# Autodesk Inventor assembly: HCMUTE-CDT23-PLXR_KHUNG
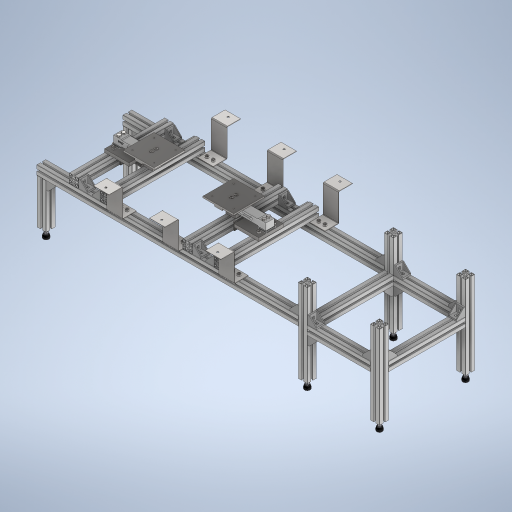
[picture p0: Inventor's stored thumbnail of the model, 512x512]
Saved by Autodesk Inventor 2023 (Build 270158000, 158)
## iProperties
Created: 2023-11-19
Part Number: HCMUTE-CDT23-PLXR_KHUNG
Document SubType Name: Assembly
Designer: havie
Mass: 52555 g
Surface Area: 83477.5 cm^2
Volume: 13075.1 cm^3
Density: 4.01946 g/cm^3
Author: havie
## Documents named in this file (13)
- D:\DO_AN_CDT\1.1. PART\HCMUTE-CDT23-PLXR_KHUNG.iam
- D:\DO_AN_CDT\1.1. PART\HCMUTE-CDT23-FRAME_ASEMBLY.iam
- C:\Users\havie\Documents\Inventor\Content Center Files\R2023\en-US\ISO 4762(2)\ISO 4762 - M6 x 16ISO.ipt
- C:\Users\havie\Documents\Inventor\Content Center Files\R2023\en-US\ISO 4762(2)\ISO 4762 - M6 x 25ISO.ipt
- D:\DO_AN_CDT\1.1. PART\HCMUTE-CDT23-LOADCELL.ipt
- D:\DO_AN_CDT\1.1. PART\HCMUTE-CDT23-DE_CHEM_LOADCELL.ipt
- D:\DO_AN_CDT\1.1. PART\HCMUTE-CDT23-DE_GA_LOADCELL.ipt
- D:\DO_AN_CDT\1.1. PART\HCMUTE-CDT23-GOI_CHONG_QTAI.ipt
- D:\DO_AN_CDT\1.1. PART\HCMUTE-CDT23-GOI_DO.ipt
- C:\Users\havie\Documents\Inventor\Content Center Files\R2023\en-US\ISO 4017(1)\ISO 4017 - M6 x 45 - ISO.ipt
- C:\Users\havie\Documents\Inventor\Content Center Files\R2023\en-US\ISO 4762(2)\ISO 4762 - M6 x 10ISO.ipt
- D:\DO_AN_CDT\1.1. PART\HCMUTE-CDT23-BAN_CAN_LOADCELL.ipt
- D:\DO_AN_CDT\1.1. PART\HCMUTE-CDT23-KXL_CHAN-GA.ipt
## Components (53 placed, 12 different names)
1. HCMUTE-CDT23-FRAME_ASEMBLY:1 [sub-assembly] — Mate:84, Flush:8, Flush:9, Mate:92, Flush:12, Mate:102, Flush:13, Mate:152, Flush:16, Mate:153, Flush:18, Mate:154, Flush:20, Mate:276, Flush:52, Mate:277, Mate:282, Mate:283, Mate:284, Mate:285, Mate:320, Flush:63, Mate:321, Mate:322, Mate:323
2. HCMUTE-CDT23-LOADCELL:1 — Mate:88, Mate:89, Mate:90, Mate:94, Mate:95, Mate:96, Mate:97, Flush:14, Mate:113, Mate:114, Mate:115
3. HCMUTE-CDT23-DE_CHEM_LOADCELL:1 — Mate:85, Mate:86, Mate:87, Mate:88, Mate:89, Mate:90
4. HCMUTE-CDT23-DE_GA_LOADCELL:1 — Mate:84, Flush:8, Flush:9, Mate:85, Mate:86, Mate:87, Mate:93, Mate:98, Mate:99, Mate:100, Mate:101, Flush:19
5. HCMUTE-CDT23-GOI_CHONG_QTAI:1 — Mate:102, Flush:13, Mate:103, Mate:104, Flush:14
6. HCMUTE-CDT23-GOI_DO:1 — Mate:92, Flush:12, Mate:93, Mate:105, Mate:106, Mate:107, Mate:108, Mate:109, Mate:110, Mate:111, Mate:112, Flush:17
7. ISO 4017 M6 x 45:1 — Mate:94, Mate:97
8. ISO 4017 M6 x 45:2 — Mate:95, Mate:96
9. ISO 4762 M6 x 16:31 — Mate:100, Mate:101
10. ISO 4762 M6 x 16:33 — Mate:98, Mate:99
11. ISO 4762 M6 x 16:34 — Mate:103, Mate:104
12. ISO 4762 M6 x 10:1 — Mate:105, Mate:106
13. ISO 4762 M6 x 10:2 — Mate:111, Mate:112
14. ISO 4762 M6 x 10:3 — Mate:109, Mate:110
15. ISO 4762 M6 x 10:4 — Mate:107, Mate:108
16. HCMUTE-CDT23-BAN_CAN_LOADCELL:1 — Mate:113, Mate:114, Mate:115, Mate:116, Mate:117, Mate:118, Mate:119
17. ISO 4762 M6 x 25:5 — Mate:116, Mate:118
18. ISO 4762 M6 x 25:6 — Mate:117, Mate:119
19. HCMUTE-CDT23-LOADCELL:2 — Flush:21
20. HCMUTE-CDT23-DE_CHEM_LOADCELL:2
21. HCMUTE-CDT23-DE_GA_LOADCELL:2 — Mate:153, Flush:18, Flush:19
22. HCMUTE-CDT23-GOI_CHONG_QTAI:2 — Mate:154, Flush:20, Flush:21
23. HCMUTE-CDT23-GOI_DO:2 — Mate:152, Flush:16, Flush:17
24. ISO 4017 M6 x 45:3
25. ISO 4017 M6 x 45:4
26. ISO 4762 M6 x 16:35
27. ISO 4762 M6 x 16:36
28. ISO 4762 M6 x 16:37
29. ISO 4762 M6 x 10:5
30. ISO 4762 M6 x 10:6
31. ISO 4762 M6 x 10:7
32. ISO 4762 M6 x 10:8
33. HCMUTE-CDT23-BAN_CAN_LOADCELL:2
34. ISO 4762 M6 x 25:7
35. ISO 4762 M6 x 25:8
36. HCMUTE-CDT23-KXL_CHAN-GA:1 — Mate:276, Flush:52, Mate:277, Mate:278, Mate:279, Mate:280, Mate:281, Flush:53
37. HCMUTE-CDT23-KXL_CHAN-GA:2 — Mate:282, Mate:283, Flush:53, Flush:54, Flush:65
38. HCMUTE-CDT23-KXL_CHAN-GA:3 — Mate:284, Mate:285, Flush:54, Flush:67
39. HCMUTE-CDT23-KXL_CHAN-GA:4 — Mate:320, Flush:63, Mate:321, Flush:64, Flush:66
40. HCMUTE-CDT23-KXL_CHAN-GA:5 — Mate:322, Flush:64, Flush:65
41. HCMUTE-CDT23-KXL_CHAN-GA:6 — Mate:323, Flush:66, Flush:67, Mate:327, Mate:328, Mate:329, Mate:330
42. ISO 4762 M6 x 10:9 — Mate:280, Mate:281
43. ISO 4762 M6 x 10:10 — Mate:278, Mate:279
44. ISO 4762 M6 x 10:11
45. ISO 4762 M6 x 10:12
46. ISO 4762 M6 x 10:13
47. ISO 4762 M6 x 10:14
48. ISO 4762 M6 x 10:16 — Mate:329, Mate:330
49. ISO 4762 M6 x 10:15 — Mate:327, Mate:328
50. ISO 4762 M6 x 10:17
51. ISO 4762 M6 x 10:18
52. ISO 4762 M6 x 10:19
53. ISO 4762 M6 x 10:20
## Component patterns: (3 elements, first: ISO 4762 M6 x 10:9 + ISO 4762 M6 x 10:10), (3 elements, first: ISO 4762 M6 x 10:16 + ISO 4762 M6 x 10:15)
## Relationships (111: Mate 89, Flush 20, Symmetry 2)
- Mate:84: HCMUTE-CDT23-FRAME_ASEMBLY:1 ↔ HCMUTE-CDT23-DE_GA_LOADCELL:1
- Flush:8: HCMUTE-CDT23-FRAME_ASEMBLY:1 ↔ HCMUTE-CDT23-DE_GA_LOADCELL:1
- Flush:9 (115 mm): HCMUTE-CDT23-FRAME_ASEMBLY:1 ↔ HCMUTE-CDT23-DE_GA_LOADCELL:1
- Mate:85: HCMUTE-CDT23-DE_CHEM_LOADCELL:1 ↔ HCMUTE-CDT23-DE_GA_LOADCELL:1
- Mate:86: HCMUTE-CDT23-DE_CHEM_LOADCELL:1 ↔ HCMUTE-CDT23-DE_GA_LOADCELL:1
- Mate:87: HCMUTE-CDT23-DE_CHEM_LOADCELL:1 ↔ HCMUTE-CDT23-DE_GA_LOADCELL:1
- Mate:88: HCMUTE-CDT23-LOADCELL:1 ↔ HCMUTE-CDT23-DE_CHEM_LOADCELL:1
- Mate:89: HCMUTE-CDT23-LOADCELL:1 ↔ HCMUTE-CDT23-DE_CHEM_LOADCELL:1
- Mate:90: HCMUTE-CDT23-LOADCELL:1 ↔ HCMUTE-CDT23-DE_CHEM_LOADCELL:1
- Mate:92: HCMUTE-CDT23-FRAME_ASEMBLY:1 ↔ HCMUTE-CDT23-GOI_DO:1
- Flush:12: HCMUTE-CDT23-FRAME_ASEMBLY:1 ↔ HCMUTE-CDT23-GOI_DO:1
- Mate:93: HCMUTE-CDT23-DE_GA_LOADCELL:1 ↔ HCMUTE-CDT23-GOI_DO:1
- Mate:94: HCMUTE-CDT23-LOADCELL:1 ↔ ISO 4017 M6 x 45:1
- Mate:95: HCMUTE-CDT23-LOADCELL:1 ↔ ISO 4017 M6 x 45:2
- Mate:96: HCMUTE-CDT23-LOADCELL:1 ↔ ISO 4017 M6 x 45:2
- Mate:97: HCMUTE-CDT23-LOADCELL:1 ↔ ISO 4017 M6 x 45:1
- Mate:98: HCMUTE-CDT23-DE_GA_LOADCELL:1 ↔ ISO 4762 M6 x 16:33
- Mate:99: HCMUTE-CDT23-DE_GA_LOADCELL:1 ↔ ISO 4762 M6 x 16:33
- Mate:100: HCMUTE-CDT23-DE_GA_LOADCELL:1 ↔ ISO 4762 M6 x 16:31
- Mate:101: HCMUTE-CDT23-DE_GA_LOADCELL:1 ↔ ISO 4762 M6 x 16:31
- Mate:102: HCMUTE-CDT23-FRAME_ASEMBLY:1 ↔ HCMUTE-CDT23-GOI_CHONG_QTAI:1
- Flush:13: HCMUTE-CDT23-FRAME_ASEMBLY:1 ↔ HCMUTE-CDT23-GOI_CHONG_QTAI:1
- Mate:103: HCMUTE-CDT23-GOI_CHONG_QTAI:1 ↔ ISO 4762 M6 x 16:34
- Mate:104: HCMUTE-CDT23-GOI_CHONG_QTAI:1 ↔ ISO 4762 M6 x 16:34
- Flush:14 (-1.5 mm): HCMUTE-CDT23-LOADCELL:1 ↔ HCMUTE-CDT23-GOI_CHONG_QTAI:1
- Mate:105: HCMUTE-CDT23-GOI_DO:1 ↔ ISO 4762 M6 x 10:1
- Mate:106: HCMUTE-CDT23-GOI_DO:1 ↔ ISO 4762 M6 x 10:1
- Mate:107: HCMUTE-CDT23-GOI_DO:1 ↔ ISO 4762 M6 x 10:4
- Mate:108: HCMUTE-CDT23-GOI_DO:1 ↔ ISO 4762 M6 x 10:4
- Mate:109: HCMUTE-CDT23-GOI_DO:1 ↔ ISO 4762 M6 x 10:3
- Mate:110: HCMUTE-CDT23-GOI_DO:1 ↔ ISO 4762 M6 x 10:3
- Mate:111: HCMUTE-CDT23-GOI_DO:1 ↔ ISO 4762 M6 x 10:2
- Mate:112: HCMUTE-CDT23-GOI_DO:1 ↔ ISO 4762 M6 x 10:2
- Mate:113: HCMUTE-CDT23-LOADCELL:1 ↔ HCMUTE-CDT23-BAN_CAN_LOADCELL:1
- Mate:114: HCMUTE-CDT23-LOADCELL:1 ↔ HCMUTE-CDT23-BAN_CAN_LOADCELL:1
- Mate:115: HCMUTE-CDT23-LOADCELL:1 ↔ HCMUTE-CDT23-BAN_CAN_LOADCELL:1
- Mate:116: HCMUTE-CDT23-BAN_CAN_LOADCELL:1 ↔ ISO 4762 M6 x 25:5
- Mate:117: HCMUTE-CDT23-BAN_CAN_LOADCELL:1 ↔ ISO 4762 M6 x 25:6
- Mate:118: HCMUTE-CDT23-BAN_CAN_LOADCELL:1 ↔ ISO 4762 M6 x 25:5
- Mate:119: HCMUTE-CDT23-BAN_CAN_LOADCELL:1 ↔ ISO 4762 M6 x 25:6
- [Mate]: HCMUTE-CDT23-DE_CHEM_LOADCELL:2 ↔ HCMUTE-CDT23-DE_GA_LOADCELL:2
- [Mate]: HCMUTE-CDT23-DE_CHEM_LOADCELL:2 ↔ HCMUTE-CDT23-DE_GA_LOADCELL:2
- [Mate]: HCMUTE-CDT23-DE_CHEM_LOADCELL:2 ↔ HCMUTE-CDT23-DE_GA_LOADCELL:2
- [Mate]: HCMUTE-CDT23-LOADCELL:2 ↔ HCMUTE-CDT23-DE_CHEM_LOADCELL:2
- [Mate]: HCMUTE-CDT23-LOADCELL:2 ↔ HCMUTE-CDT23-DE_CHEM_LOADCELL:2
- [Mate]: HCMUTE-CDT23-LOADCELL:2 ↔ HCMUTE-CDT23-DE_CHEM_LOADCELL:2
- [Mate]: HCMUTE-CDT23-DE_GA_LOADCELL:2 ↔ HCMUTE-CDT23-GOI_DO:2
- [Mate]: HCMUTE-CDT23-LOADCELL:2 ↔ ISO 4017 M6 x 45:3
- [Mate]: HCMUTE-CDT23-LOADCELL:2 ↔ ISO 4017 M6 x 45:4
- [Mate]: HCMUTE-CDT23-LOADCELL:2 ↔ ISO 4017 M6 x 45:4
- [Mate]: HCMUTE-CDT23-LOADCELL:2 ↔ ISO 4017 M6 x 45:3
- [Mate]: HCMUTE-CDT23-DE_GA_LOADCELL:2 ↔ ISO 4762 M6 x 16:36
- [Mate]: HCMUTE-CDT23-DE_GA_LOADCELL:2 ↔ ISO 4762 M6 x 16:36
- [Mate]: HCMUTE-CDT23-DE_GA_LOADCELL:2 ↔ ISO 4762 M6 x 16:35
- [Mate]: HCMUTE-CDT23-DE_GA_LOADCELL:2 ↔ ISO 4762 M6 x 16:35
- [Mate]: HCMUTE-CDT23-GOI_CHONG_QTAI:2 ↔ ISO 4762 M6 x 16:37
- [Mate]: HCMUTE-CDT23-GOI_CHONG_QTAI:2 ↔ ISO 4762 M6 x 16:37
- [Flush] (-1.5 mm): HCMUTE-CDT23-LOADCELL:2 ↔ HCMUTE-CDT23-GOI_CHONG_QTAI:2
- [Mate]: HCMUTE-CDT23-GOI_DO:2 ↔ ISO 4762 M6 x 10:5
- [Mate]: HCMUTE-CDT23-GOI_DO:2 ↔ ISO 4762 M6 x 10:5
- [Mate]: HCMUTE-CDT23-GOI_DO:2 ↔ ISO 4762 M6 x 10:8
- [Mate]: HCMUTE-CDT23-GOI_DO:2 ↔ ISO 4762 M6 x 10:8
- [Mate]: HCMUTE-CDT23-GOI_DO:2 ↔ ISO 4762 M6 x 10:7
- [Mate]: HCMUTE-CDT23-GOI_DO:2 ↔ ISO 4762 M6 x 10:7
- [Mate]: HCMUTE-CDT23-GOI_DO:2 ↔ ISO 4762 M6 x 10:6
- [Mate]: HCMUTE-CDT23-GOI_DO:2 ↔ ISO 4762 M6 x 10:6
- [Mate]: HCMUTE-CDT23-LOADCELL:2 ↔ HCMUTE-CDT23-BAN_CAN_LOADCELL:2
- [Mate]: HCMUTE-CDT23-LOADCELL:2 ↔ HCMUTE-CDT23-BAN_CAN_LOADCELL:2
- [Mate]: HCMUTE-CDT23-LOADCELL:2 ↔ HCMUTE-CDT23-BAN_CAN_LOADCELL:2
- [Mate]: HCMUTE-CDT23-BAN_CAN_LOADCELL:2 ↔ ISO 4762 M6 x 25:7
- [Mate]: HCMUTE-CDT23-BAN_CAN_LOADCELL:2 ↔ ISO 4762 M6 x 25:8
- [Mate]: HCMUTE-CDT23-BAN_CAN_LOADCELL:2 ↔ ISO 4762 M6 x 25:7
- [Mate]: HCMUTE-CDT23-BAN_CAN_LOADCELL:2 ↔ ISO 4762 M6 x 25:8
- Mate:152: HCMUTE-CDT23-FRAME_ASEMBLY:1 ↔ HCMUTE-CDT23-GOI_DO:2
- Flush:16: HCMUTE-CDT23-FRAME_ASEMBLY:1 ↔ HCMUTE-CDT23-GOI_DO:2
- Flush:17: HCMUTE-CDT23-GOI_DO:1 ↔ HCMUTE-CDT23-GOI_DO:2
- Mate:153: HCMUTE-CDT23-FRAME_ASEMBLY:1 ↔ HCMUTE-CDT23-DE_GA_LOADCELL:2
- Flush:18: HCMUTE-CDT23-FRAME_ASEMBLY:1 ↔ HCMUTE-CDT23-DE_GA_LOADCELL:2
- Flush:19: HCMUTE-CDT23-DE_GA_LOADCELL:1 ↔ HCMUTE-CDT23-DE_GA_LOADCELL:2
- Mate:154: HCMUTE-CDT23-FRAME_ASEMBLY:1 ↔ HCMUTE-CDT23-GOI_CHONG_QTAI:2
- Flush:20: HCMUTE-CDT23-FRAME_ASEMBLY:1 ↔ HCMUTE-CDT23-GOI_CHONG_QTAI:2
- Flush:21 (-1.5 mm): HCMUTE-CDT23-LOADCELL:2 ↔ HCMUTE-CDT23-GOI_CHONG_QTAI:2
- Symmetry:1
- Symmetry:2
- Mate:235
- Mate:276: HCMUTE-CDT23-FRAME_ASEMBLY:1 ↔ HCMUTE-CDT23-KXL_CHAN-GA:1
- Flush:52 (-15 mm): HCMUTE-CDT23-FRAME_ASEMBLY:1 ↔ HCMUTE-CDT23-KXL_CHAN-GA:1
- Mate:277: HCMUTE-CDT23-FRAME_ASEMBLY:1 ↔ HCMUTE-CDT23-KXL_CHAN-GA:1
- Mate:278: HCMUTE-CDT23-KXL_CHAN-GA:1 ↔ ISO 4762 M6 x 10:10
- Mate:279: HCMUTE-CDT23-KXL_CHAN-GA:1 ↔ ISO 4762 M6 x 10:10
- Mate:280: HCMUTE-CDT23-KXL_CHAN-GA:1 ↔ ISO 4762 M6 x 10:9
- Mate:281: HCMUTE-CDT23-KXL_CHAN-GA:1 ↔ ISO 4762 M6 x 10:9
- Mate:282: HCMUTE-CDT23-FRAME_ASEMBLY:1 ↔ HCMUTE-CDT23-KXL_CHAN-GA:2
- Mate:283: HCMUTE-CDT23-FRAME_ASEMBLY:1 ↔ HCMUTE-CDT23-KXL_CHAN-GA:2
- Flush:53: HCMUTE-CDT23-KXL_CHAN-GA:1 ↔ HCMUTE-CDT23-KXL_CHAN-GA:2
- Mate:284 (6 mm): HCMUTE-CDT23-FRAME_ASEMBLY:1 ↔ HCMUTE-CDT23-KXL_CHAN-GA:3
- Mate:285: HCMUTE-CDT23-FRAME_ASEMBLY:1 ↔ HCMUTE-CDT23-KXL_CHAN-GA:3
- Flush:54: HCMUTE-CDT23-KXL_CHAN-GA:2 ↔ HCMUTE-CDT23-KXL_CHAN-GA:3
- Mate:320: HCMUTE-CDT23-FRAME_ASEMBLY:1 ↔ HCMUTE-CDT23-KXL_CHAN-GA:4
- Flush:63 (-16 mm): HCMUTE-CDT23-FRAME_ASEMBLY:1 ↔ HCMUTE-CDT23-KXL_CHAN-GA:4
- Mate:321: HCMUTE-CDT23-FRAME_ASEMBLY:1 ↔ HCMUTE-CDT23-KXL_CHAN-GA:4
- Mate:322: HCMUTE-CDT23-FRAME_ASEMBLY:1 ↔ HCMUTE-CDT23-KXL_CHAN-GA:5
- Flush:64: HCMUTE-CDT23-KXL_CHAN-GA:4 ↔ HCMUTE-CDT23-KXL_CHAN-GA:5
- Flush:65: HCMUTE-CDT23-KXL_CHAN-GA:2 ↔ HCMUTE-CDT23-KXL_CHAN-GA:5
- Mate:323: HCMUTE-CDT23-FRAME_ASEMBLY:1 ↔ HCMUTE-CDT23-KXL_CHAN-GA:6
- Flush:66: HCMUTE-CDT23-KXL_CHAN-GA:4 ↔ HCMUTE-CDT23-KXL_CHAN-GA:6
- Flush:67: HCMUTE-CDT23-KXL_CHAN-GA:3 ↔ HCMUTE-CDT23-KXL_CHAN-GA:6
- Mate:327: HCMUTE-CDT23-KXL_CHAN-GA:6 ↔ ISO 4762 M6 x 10:15
- Mate:328: HCMUTE-CDT23-KXL_CHAN-GA:6 ↔ ISO 4762 M6 x 10:15
- Mate:329: HCMUTE-CDT23-KXL_CHAN-GA:6 ↔ ISO 4762 M6 x 10:16
- Mate:330: HCMUTE-CDT23-KXL_CHAN-GA:6 ↔ ISO 4762 M6 x 10:16
## Named parameters: d151_d112 = 0 mm, d152_d113 = 0 mm, d153_d114 = 0 mm, d154_d115 = 0 mm, d155_d121 = 0 mm, d156_d122 = 0 mm, d157_d123 = 0 mm, d158_d124 = 0 mm, d159_d110 = 0 mm, d160_d111 = 0 mm, d161_d125 = 0 mm, d162_d126 = 0 mm, d163_d127 = 0 mm, d164_d128 = 0 mm, d165_d129 = 0 mm, d166_d133 = 0 mm, d167_d134 = 0 mm, d168_d135 = -1.5 mm, d169_d149 = 0 mm, d170_d150 = 0 mm, d171_d136 = 0 mm, d172_d137 = 0 mm, d173_d138 = 0 mm, d174_d139 = 0 mm, d175_d140 = 0 mm, d176_d141 = 0 mm, d177_d142 = 0 mm, d178_d143 = 0 mm, d179_d144 = 0 mm, d180_d145 = 0 mm, d181_d146 = 0 mm, d182_d147 = 0 mm, d183_d148 = 0 mm
